# Autodesk Inventor assembly: escconnector
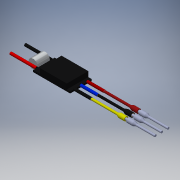
[picture p0: Inventor's stored thumbnail of the model, 180x180]
Saved by Autodesk Inventor 2016 (Build 200138000, 138)
## iProperties
Created: 2014-11-30
Part Number: escconnector
Document SubType Name: Assembly
Designer: Admin
Sending System: SolidWorks 2014
Last Author: pietrooo
Last Saved: 2014-11-30
Author: Admin
## Documents named in this file (8)
- E:\Documents\GITHUB\Side-Projects\Quadcopter\escconnector.iam
- E:\Downloads\esc connector\wirefemaleyellow.ipt
- E:\Downloads\esc connector\wirefemalered.ipt
- E:\Downloads\esc connector\wirefemaleblack.ipt
- E:\Downloads\esc connector\wiremaleyellow.ipt
- E:\Downloads\esc connector\wiremaleblack.ipt
- E:\Downloads\esc connector\wiremalered.ipt
- E:\Documents\GITHUB\Side-Projects\Quadcopter\esc.ipt
## Components (7 placed, 7 different names)
1. wirefemaleyellow:1 — Mate:1, Mate:4
2. wirefemalered:1 — Mate:3, Mate:6
3. wirefemaleblack:1 — Mate:2, Mate:5
4. wiremaleyellow:1 — Mate:4
5. wiremaleblack:1 — Mate:5
6. wiremalered:1 — Mate:6
7. esc:1 — Mate:1, Mate:2, Mate:3
## Relationships (6: Mate 6)
- Mate:1: wirefemaleyellow:1 ↔ esc:1
- Mate:2: wirefemaleblack:1 ↔ esc:1
- Mate:3: wirefemalered:1 ↔ esc:1
- Mate:4: wirefemaleyellow:1 ↔ wiremaleyellow:1
- Mate:5: wirefemaleblack:1 ↔ wiremaleblack:1
- Mate:6: wirefemalered:1 ↔ wiremalered:1
